# Autodesk Inventor assembly: HbSensorU02
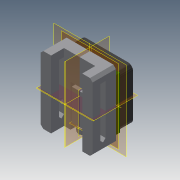
[picture p0: Inventor's stored thumbnail of the model, 180x180]
Saved by Autodesk Inventor 2015 SP1 (Build 190203100, 203)
## iProperties
Created: 2016-01-28
Part Number: HbSensorU02
Document SubType Name: Assembly
Designer: Yamaura
Author: Yamaura
## Documents named in this file (6)
- C:\Users\Yamaura\Documents\GitHub\HACKberry\HACKberry-hardware\3D\Inventor\Parts\HbSensorU02.iam
- C:\Users\Yamaura\Documents\GitHub\HACKberry\HACKberry-hardware\3D\Inventor\Parts\HbSensorBoard02.ipt
- C:\Users\Yamaura\Documents\GitHub\HACKberry\HACKberry-hardware\3D\Inventor\Parts\HbSensorHolder02.ipt
- C:\Users\Yamaura\Documents\GitHub\HACKberry\HACKberry-hardware\3D\Inventor\Parts\ST-PJ-312.ipt
- C:\Users\Yamaura\Documents\GitHub\HACKberry\HACKberry-hardware\3D\Inventor\Parts\HbSensorCushion02.ipt
- C:\Users\Yamaura\Documents\GitHub\HACKberry\HACKberry-hardware\3D\Inventor\Parts\QRE1113GR.ipt
## Components (5 placed, 5 different names)
1. HbSensorBoard02:1 — メイト:1, メイト:2, メイト:3, メイト:4, メイト:5, メイト:8, メイト:10
2. HbSensorHolder02:1 — メイト:1, メイト:2, メイト:3
3. ST-PJ-312:1 — メイト:4, メイト:5, メイト:6
4. HbSensorCushion02:1 — メイト:7, メイト:8, メイト:9
5. QRE1113GR:1 — メイト:10, メイト:11, メイト:12
## Relationships (12: Mate 12)
- メイト:1 [Mate]: HbSensorBoard02:1 ↔ HbSensorHolder02:1
- メイト:2 [Mate]: HbSensorBoard02:1 ↔ HbSensorHolder02:1
- メイト:3 [Mate]: HbSensorBoard02:1 ↔ HbSensorHolder02:1
- メイト:4 [Mate]: HbSensorBoard02:1 ↔ ST-PJ-312:1
- メイト:5 [Mate]: HbSensorBoard02:1 ↔ ST-PJ-312:1
- メイト:6 [Mate]: ST-PJ-312:1
- メイト:7 [Mate]: HbSensorCushion02:1
- メイト:8 [Mate]: HbSensorBoard02:1 ↔ HbSensorCushion02:1
- メイト:9 [Mate]: HbSensorCushion02:1
- メイト:10 [Mate]: HbSensorBoard02:1 ↔ QRE1113GR:1
- メイト:11 [Mate]: QRE1113GR:1
- メイト:12 [Mate]: QRE1113GR:1
